# Autodesk Inventor assembly: Baugruppe6
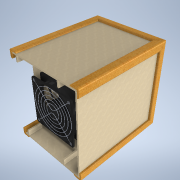
[picture p0: Inventor's stored thumbnail of the model, 180x180]
Saved by Autodesk Inventor 2020 (Build 240168000, 168)
## iProperties
Created: 2022-03-23
Part Number: Baugruppe6
Document SubType Name: Assembly
Designer: Eric
Author: Eric
## Documents named in this file (19)
- C:\Users\Eric\Documents\Projekte\NAS\Baugruppe6.iam
- C:\Users\Eric\Documents\Projekte\NAS\gigabyte b360n wifi.iam
- C:\Users\Eric\Documents\Projekte\NAS\pcie 4x splitter step.iam
- C:\Users\Eric\Documents\Projekte\NAS\pico_PSU.ipt
- C:\Users\Eric\Documents\Projekte\NAS\HDD_SATA_3.5.ipt
- C:\Users\Eric\Documents\Projekte\NAS\Platte1.ipt
- C:\Users\Eric\Documents\Projekte\NAS\Platte2.ipt
- C:\Users\Eric\Documents\Projekte\NAS\sideHolder.ipt
- C:\Users\Eric\Documents\Projekte\NAS\120mm Fan.ipt
- C:\Users\Eric\Documents\Projekte\NAS\io_shield.ipt
- C:\Users\Eric\Documents\Projekte\NAS\Querstrebe.ipt
- C:\Users\Eric\Documents\Projekte\NAS\Querstrebe2.ipt
- C:\Users\Eric\Documents\Projekte\NAS\Seitenplatte.ipt
- C:\Users\Eric\Documents\Projekte\NAS\eckeHochkant.ipt
- C:\Users\Eric\Documents\Projekte\NAS\frontPlatte.ipt
- C:\Users\Eric\Documents\Projekte\NAS\backPlatte.ipt
- C:\Users\Eric\Documents\Projekte\NAS\winkelTop.ipt
- C:\Users\Eric\Documents\Projekte\NAS\winkelTop2.ipt
- C:\Users\Eric\Documents\Projekte\NAS\topPlatte.ipt
## Components (35 placed, 18 different names)
1. gigabyte b360n wifi:1 [sub-assembly] — Passend:1, Passend:2, Winkel:1, Passend:3, Passend:4, Passend:5, Passend:13, Fluchtend:26, Passend:27, Passend:36, Winkel:2, Passend:61, Passend:62
2. pcie 4x splitter step:1 [sub-assembly] — Passend:1, Passend:2, Winkel:1
3. pico_PSU:1 — Passend:3, Passend:4, Passend:5
4. HDD_SATA_3.5:1 — Fluchtend:1, Fluchtend:2, Fluchtend:5, Fluchtend:8, Fluchtend:9
5. HDD_SATA_3.5:2 — Fluchtend:1, Fluchtend:6, Fluchtend:7, Fluchtend:8
6. HDD_SATA_3.5:3 — Fluchtend:3, Fluchtend:4, Fluchtend:5, Fluchtend:9, Passend:21, Passend:33, Passend:34
7. HDD_SATA_3.5:4 — Fluchtend:2, Fluchtend:3, Fluchtend:4, Fluchtend:6, Fluchtend:7, Fluchtend:11, Fluchtend:12, Fluchtend:15
8. HDD_SATA_3.5:5 — Fluchtend:11, Fluchtend:12, Fluchtend:13, Fluchtend:14, Fluchtend:15, Fluchtend:16
9. HDD_SATA_3.5:6 — Fluchtend:13, Fluchtend:14, Fluchtend:16
10. Platte1:1 — Passend:8, Passend:21, Passend:22, Fluchtend:24, Passend:28, Passend:29, Passend:33, Passend:34, Passend:39, Passend:40, Passend:47, Fluchtend:35, Passend:50
11. Platte2:1 — Passend:9, Passend:10, Passend:13, Fluchtend:25, Fluchtend:26, Passend:35, Passend:37, Passend:38, Fluchtend:31
12. sideHolder:1 — Passend:8, Passend:9, Passend:10, Passend:22, Fluchtend:23, Passend:23, Passend:26, Passend:27, Passend:40, Passend:41, Fluchtend:29, Passend:46, Fluchtend:36, Fluchtend:40
13. Platte1:2 — Passend:23, Passend:24, Passend:25, Passend:26, Fluchtend:24, Fluchtend:25, Passend:30, Passend:31, Fluchtend:39
14. 120mm Fan:1 — Passend:35, Passend:37, Passend:38
15. sideHolder:4 — Fluchtend:23, Passend:24, Passend:25, Passend:44
16. sideHolder:5 — Passend:28, Passend:30, Fluchtend:27, Passend:42, Fluchtend:28, Fluchtend:38
17. sideHolder:6 — Passend:29, Passend:31, Fluchtend:27, Passend:39
18. io_shield:1 — Passend:36, Winkel:2, Passend:61, Passend:62
19. Querstrebe:1 — Passend:42, Fluchtend:28, Fluchtend:30, Fluchtend:31, Passend:43, Fluchtend:32
20. Querstrebe:2 — Passend:41, Fluchtend:29, Fluchtend:30, Passend:45, Fluchtend:33
21. Querstrebe2:1 — Passend:43, Passend:44, Fluchtend:32
22. Querstrebe2:2 — Passend:45, Passend:46, Fluchtend:33
23. Seitenplatte:1 — Passend:47, Fluchtend:35, Fluchtend:36, Passend:48, Fluchtend:37, Passend:49, Passend:55, Fluchtend:42, Fluchtend:44, Passend:63, Passend:64
24. eckeHochkant:1 — Passend:48, Fluchtend:37, Passend:49, Passend:51, Passend:52, Passend:65
25. Seitenplatte:2 — Passend:50, Fluchtend:38, Fluchtend:39, Passend:54, Fluchtend:43, Passend:56, Passend:60, Passend:69
26. frontPlatte:1 — Passend:51, Fluchtend:40, Passend:52, Passend:53, Fluchtend:41, Passend:73
27. eckeHochkant:2 — Passend:55, Fluchtend:42, Passend:57, Passend:71
28. eckeHochkant:3 — Passend:53, Fluchtend:41, Passend:54, Passend:74
29. eckeHochkant:4 — Fluchtend:43, Passend:56, Passend:58, Passend:59, Passend:68
30. backPlatte:1 — Passend:57, Fluchtend:44, Passend:58, Passend:59, Passend:60, Passend:70, Passend:76
31. winkelTop:1 — Passend:63, Passend:64, Passend:65, Fluchtend:45, Passend:72
32. winkelTop:3 — Passend:68, Passend:69, Fluchtend:45, Passend:75, Passend:78
33. winkelTop2:1 — Passend:73, Passend:74, Passend:75, Passend:77
34. winkelTop2:2 — Passend:70, Passend:71, Passend:72
35. topPlatte:1 — Passend:76, Passend:77, Passend:78
## Relationships (103: Mate 64, Flush 37, Angle 2)
- Passend:1 [Mate]: gigabyte b360n wifi:1 ↔ pcie 4x splitter step:1
- Passend:2 [Mate]: gigabyte b360n wifi:1 ↔ pcie 4x splitter step:1
- Winkel:1 [Angle] (0 deg): gigabyte b360n wifi:1 ↔ pcie 4x splitter step:1
- Passend:3 [Mate]: gigabyte b360n wifi:1 ↔ pico_PSU:1
- Passend:4 [Mate]: gigabyte b360n wifi:1 ↔ pico_PSU:1
- Passend:5 [Mate]: gigabyte b360n wifi:1 ↔ pico_PSU:1
- Fluchtend:1 [Flush]: HDD_SATA_3.5:1 ↔ HDD_SATA_3.5:2
- Fluchtend:2 [Flush]: HDD_SATA_3.5:1 ↔ HDD_SATA_3.5:4
- Fluchtend:3 [Flush]: HDD_SATA_3.5:3 ↔ HDD_SATA_3.5:4
- Fluchtend:4 [Flush]: HDD_SATA_3.5:3 ↔ HDD_SATA_3.5:4
- Fluchtend:5 [Flush]: HDD_SATA_3.5:1 ↔ HDD_SATA_3.5:3
- Fluchtend:6 [Flush]: HDD_SATA_3.5:2 ↔ HDD_SATA_3.5:4
- Fluchtend:7 [Flush] (30 mm): HDD_SATA_3.5:2 ↔ HDD_SATA_3.5:4
- Fluchtend:8 [Flush] (30 mm): HDD_SATA_3.5:1 ↔ HDD_SATA_3.5:2
- Fluchtend:9 [Flush] (-30 mm): HDD_SATA_3.5:1 ↔ HDD_SATA_3.5:3
- Fluchtend:11 [Flush]: HDD_SATA_3.5:4 ↔ HDD_SATA_3.5:5
- Fluchtend:12 [Flush] (30 mm): HDD_SATA_3.5:4 ↔ HDD_SATA_3.5:5
- Fluchtend:13 [Flush]: HDD_SATA_3.5:5 ↔ HDD_SATA_3.5:6
- Fluchtend:14 [Flush] (30 mm): HDD_SATA_3.5:5 ↔ HDD_SATA_3.5:6
- Fluchtend:15 [Flush]: HDD_SATA_3.5:4 ↔ HDD_SATA_3.5:5
- Fluchtend:16 [Flush]: HDD_SATA_3.5:5 ↔ HDD_SATA_3.5:6
- Passend:8 [Mate]: Platte1:1 ↔ sideHolder:1
- Passend:9 [Mate]: Platte2:1 ↔ sideHolder:1
- Passend:10 [Mate]: Platte2:1 ↔ sideHolder:1
- Passend:13 [Mate] (10 mm): gigabyte b360n wifi:1 ↔ Platte2:1
- Passend:21 [Mate]: HDD_SATA_3.5:3 ↔ Platte1:1
- Passend:22 [Mate]: Platte1:1 ↔ sideHolder:1
- Fluchtend:23 [Flush]: sideHolder:1 ↔ sideHolder:4
- Passend:23 [Mate]: sideHolder:1 ↔ Platte1:2
- Passend:24 [Mate]: Platte1:2 ↔ sideHolder:4
- Passend:25 [Mate]: Platte1:2 ↔ sideHolder:4
- Passend:26 [Mate]: sideHolder:1 ↔ Platte1:2
- Fluchtend:24 [Flush]: Platte1:1 ↔ Platte1:2
- Fluchtend:25 [Flush]: Platte2:1 ↔ Platte1:2
- Fluchtend:26 [Flush]: gigabyte b360n wifi:1 ↔ Platte2:1
- Passend:27 [Mate] (3 mm): gigabyte b360n wifi:1 ↔ sideHolder:1
- Passend:28 [Mate]: Platte1:1 ↔ sideHolder:5
- Passend:29 [Mate]: Platte1:1 ↔ sideHolder:6
- Passend:30 [Mate]: Platte1:2 ↔ sideHolder:5
- Passend:31 [Mate]: Platte1:2 ↔ sideHolder:6
- Fluchtend:27 [Flush]: sideHolder:5 ↔ sideHolder:6
- Passend:33 [Mate]: HDD_SATA_3.5:3 ↔ Platte1:1
- Passend:34 [Mate]: HDD_SATA_3.5:3 ↔ Platte1:1
- Passend:35 [Mate]: Platte2:1 ↔ 120mm Fan:1
- Passend:36 [Mate]: gigabyte b360n wifi:1 ↔ io_shield:1
- Winkel:2 [Angle] (90 deg): gigabyte b360n wifi:1 ↔ io_shield:1
- Passend:37 [Mate]: Platte2:1 ↔ 120mm Fan:1
- Passend:38 [Mate]: Platte2:1 ↔ 120mm Fan:1
- Passend:39 [Mate]: Platte1:1 ↔ sideHolder:6
- Passend:40 [Mate]: Platte1:1 ↔ sideHolder:1
- Passend:41 [Mate]: sideHolder:1 ↔ Querstrebe:2
- Passend:42 [Mate]: sideHolder:5 ↔ Querstrebe:1
- Fluchtend:28 [Flush]: sideHolder:5 ↔ Querstrebe:1
- Fluchtend:29 [Flush]: sideHolder:1 ↔ Querstrebe:2
- Fluchtend:30 [Flush]: Querstrebe:1 ↔ Querstrebe:2
- Fluchtend:31 [Flush]: Platte2:1 ↔ Querstrebe:1
- Passend:43 [Mate]: Querstrebe:1 ↔ Querstrebe2:1
- Passend:44 [Mate]: sideHolder:4 ↔ Querstrebe2:1
- Fluchtend:32 [Flush]: Querstrebe:1 ↔ Querstrebe2:1
- Passend:45 [Mate]: Querstrebe:2 ↔ Querstrebe2:2
- Passend:46 [Mate]: sideHolder:1 ↔ Querstrebe2:2
- Fluchtend:33 [Flush]: Querstrebe:2 ↔ Querstrebe2:2
- Passend:47 [Mate]: Platte1:1 ↔ Seitenplatte:1
- Fluchtend:35 [Flush]: Platte1:1 ↔ Seitenplatte:1
- Fluchtend:36 [Flush]: sideHolder:1 ↔ Seitenplatte:1
- Passend:48 [Mate]: Seitenplatte:1 ↔ eckeHochkant:1
- Fluchtend:37 [Flush]: Seitenplatte:1 ↔ eckeHochkant:1
- Passend:49 [Mate] (4 mm): Seitenplatte:1 ↔ eckeHochkant:1
- Passend:50 [Mate]: Platte1:1 ↔ Seitenplatte:2
- Fluchtend:38 [Flush]: sideHolder:5 ↔ Seitenplatte:2
- Fluchtend:39 [Flush]: Platte1:2 ↔ Seitenplatte:2
- Passend:51 [Mate]: eckeHochkant:1 ↔ frontPlatte:1
- Fluchtend:40 [Flush]: sideHolder:1 ↔ frontPlatte:1
- Passend:52 [Mate]: eckeHochkant:1 ↔ frontPlatte:1
- Passend:53 [Mate]: frontPlatte:1 ↔ eckeHochkant:3
- Fluchtend:41 [Flush]: frontPlatte:1 ↔ eckeHochkant:3
- Passend:54 [Mate]: Seitenplatte:2 ↔ eckeHochkant:3
- Passend:55 [Mate]: Seitenplatte:1 ↔ eckeHochkant:2
- Fluchtend:42 [Flush]: Seitenplatte:1 ↔ eckeHochkant:2
- Fluchtend:43 [Flush]: Seitenplatte:2 ↔ eckeHochkant:4
- Passend:56 [Mate]: Seitenplatte:2 ↔ eckeHochkant:4
- Passend:57 [Mate]: eckeHochkant:2 ↔ backPlatte:1
- Fluchtend:44 [Flush]: Seitenplatte:1 ↔ backPlatte:1
- Passend:58 [Mate]: eckeHochkant:4 ↔ backPlatte:1
- Passend:59 [Mate]: eckeHochkant:4 ↔ backPlatte:1
- Passend:60 [Mate]: Seitenplatte:2 ↔ backPlatte:1
- Passend:61 [Mate] (-13.27 mm): gigabyte b360n wifi:1 ↔ io_shield:1
- Passend:62 [Mate] (3.4 mm): gigabyte b360n wifi:1 ↔ io_shield:1
- Passend:63 [Mate]: Seitenplatte:1 ↔ winkelTop:1
- Passend:64 [Mate] (4 mm): Seitenplatte:1 ↔ winkelTop:1
- Passend:65 [Mate]: eckeHochkant:1 ↔ winkelTop:1
- Passend:68 [Mate]: eckeHochkant:4 ↔ winkelTop:3
- Passend:69 [Mate]: Seitenplatte:2 ↔ winkelTop:3
- Fluchtend:45 [Flush]: winkelTop:1 ↔ winkelTop:3
- Passend:70 [Mate]: backPlatte:1 ↔ winkelTop2:2
- Passend:71 [Mate]: eckeHochkant:2 ↔ winkelTop2:2
- Passend:72 [Mate]: winkelTop:1 ↔ winkelTop2:2
- Passend:73 [Mate]: frontPlatte:1 ↔ winkelTop2:1
- Passend:74 [Mate]: eckeHochkant:3 ↔ winkelTop2:1
- Passend:75 [Mate]: winkelTop:3 ↔ winkelTop2:1
- Passend:76 [Mate]: backPlatte:1 ↔ topPlatte:1
- Passend:77 [Mate]: winkelTop2:1 ↔ topPlatte:1
- Passend:78 [Mate]: winkelTop:3 ↔ topPlatte:1
